# Autodesk Inventor assembly: Final assemply edit 2
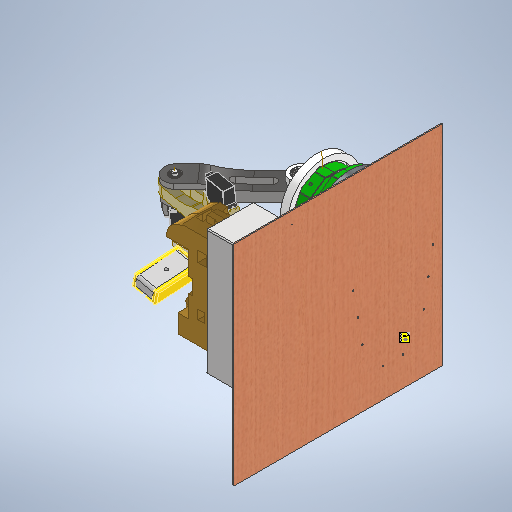
[picture p0: Inventor's stored thumbnail of the model, 512x512]
Saved by Autodesk Inventor 2025.2 (Build 292293000, 293)
## iProperties
Created: 2025-04-03
Part Number: Final assemply edit 2
Document SubType Name: Assembly
Designer: abdal
Author: abdal
## Documents named in this file (47)
- C:\Users\abdal\Desktop\FINAL MECHANICAL MOVMENT WITH STAND\Final assemply edit 2.iam
- C:\Users\abdal\Desktop\FINAL MECHANICAL MOVMENT WITH STAND\Link two .ipt
- C:\Users\abdal\Desktop\FINAL MECHANICAL MOVMENT WITH STAND\JIS B 1521 - 6800 10x19x5x1.72.ipt
- C:\Users\abdal\Desktop\FINAL MECHANICAL MOVMENT WITH STAND\DIN 472 - 19 x 1.ipt
- C:\Users\abdal\Desktop\FINAL MECHANICAL MOVMENT WITH STAND\Shaft between link2 and 3.ipt
- C:\Users\abdal\Desktop\FINAL MECHANICAL MOVMENT WITH STAND\DIN 471 - 10x1.ipt
- C:\Users\abdal\Desktop\FINAL MECHANICAL MOVMENT WITH STAND\Servo MG996R.ipt
- C:\Users\abdal\Desktop\FINAL MECHANICAL MOVMENT WITH STAND\Tower Pro MG90S Micro servo.ipt
- C:\Users\abdal\Desktop\FINAL MECHANICAL MOVMENT WITH STAND\Link Three .ipt
- C:\Users\abdal\Desktop\FINAL MECHANICAL MOVMENT WITH STAND\Link one1 .ipt
- C:\Users\abdal\Desktop\FINAL MECHANICAL MOVMENT WITH STAND\New End effector.ipt
- C:\Users\abdal\Desktop\FINAL MECHANICAL MOVMENT WITH STAND\Bidirectional shoulder.ipt
- C:\Users\abdal\Desktop\FINAL MECHANICAL MOVMENT WITH STAND\Rotating Plate edited.ipt
- C:\Users\abdal\Desktop\FINAL MECHANICAL MOVMENT WITH STAND\shatft extension.ipt
- C:\Users\abdal\Desktop\FINAL MECHANICAL MOVMENT WITH STAND\BS 292 Part 1 - 6001 - 12 x 28 x 8.ipt
- C:\Users\abdal\Desktop\FINAL MECHANICAL MOVMENT WITH STAND\DIN 471 - 12x1.ipt
- C:\Users\abdal\Desktop\FINAL MECHANICAL MOVMENT WITH STAND\DIN 472 - 28 x 1.5.ipt
- C:\Users\abdal\Desktop\FINAL MECHANICAL MOVMENT WITH STAND\Servo Horns.ipt
- C:\Users\abdal\Desktop\FINAL MECHANICAL MOVMENT WITH STAND\Printed Horn.ipt
- C:\Users\abdal\Desktop\FINAL MECHANICAL MOVMENT WITH STAND\JGY-370-1285_Motor_Assembly.ipt
- C:\Users\abdal\Desktop\FINAL MECHANICAL MOVMENT WITH STAND\Camera.ipt
- C:\Users\abdal\Desktop\FINAL MECHANICAL MOVMENT WITH STAND\BS 4174 - Type AB. No. 4 x 19 mm(1).ipt
- C:\Users\abdal\Desktop\FINAL MECHANICAL MOVMENT WITH STAND\BS 4174 - Type AB. No. 4 x 13 mm(1).ipt
- C:\Users\abdal\Desktop\FINAL MECHANICAL MOVMENT WITH STAND\BS 4174 - Type AB. No. 4 x 25 mm(1).ipt
- C:\Users\abdal\Desktop\FINAL MECHANICAL MOVMENT WITH STAND\scaled2.ipt
- C:\Users\abdal\Desktop\FINAL MECHANICAL MOVMENT WITH STAND\BASE.ipt
- C:\Users\abdal\Desktop\FINAL MECHANICAL MOVMENT WITH STAND\SHAFT.ipt
- C:\Users\abdal\Desktop\FINAL MECHANICAL MOVMENT WITH STAND\BS 5989_ Part 1 - 0 70 - 60x75x7.ipt
- C:\Users\abdal\Desktop\FINAL MECHANICAL MOVMENT WITH STAND\AS 1111 - M6 x 30.ipt
- C:\Users\abdal\Desktop\FINAL MECHANICAL MOVMENT WITH STAND\AS 1110 - M6 x 20.ipt
- C:\Users\abdal\Desktop\FINAL MECHANICAL MOVMENT WITH STAND\ANSI B18.2.4.2M - M6x1 - 10.ipt
- C:\Users\abdal\Desktop\FINAL MECHANICAL MOVMENT WITH STAND\AS 1427 - M2.5 x 12(5) I.ipt
- C:\Users\abdal\Desktop\FINAL MECHANICAL MOVMENT WITH STAND\holder for motor.ipt
- C:\Users\abdal\Desktop\FINAL MECHANICAL MOVMENT WITH STAND\DC Motor.ipt
- C:\Users\abdal\Desktop\FINAL MECHANICAL MOVMENT WITH STAND\Arduino_Mega.ipt
- C:\Users\abdal\Desktop\FINAL MECHANICAL MOVMENT WITH STAND\Breadboard Half.ipt
- C:\Users\abdal\Desktop\FINAL MECHANICAL MOVMENT WITH STAND\H-brug.ipt
- C:\Users\abdal\Documents\Inventor\Content Center Files\R2025\en-US\BS 4183(2)\BS 4183 - M3 x 7(1) I.ipt
- C:\Users\abdal\Documents\Inventor\Content Center Files\R2025\en-US\BS 4183(2)\BS 4183 - M2.5 x 5(1) I.ipt
- C:\Users\abdal\Desktop\FINAL MECHANICAL MOVMENT WITH STAND\Product stand .ipt
- C:\Users\abdal\Documents\Inventor\Content Center Files\R2025\en-US\BS 4183(2)\BS 4183 - M5 x 20(1) I.ipt
- C:\Users\abdal\Desktop\FINAL MECHANICAL MOVMENT WITH STAND\plate .ipt
- C:\Users\abdal\Desktop\FINAL MECHANICAL MOVMENT WITH STAND\L joint .ipt
- C:\Users\abdal\Desktop\FINAL MECHANICAL MOVMENT WITH STAND\L joint _MIR.ipt
- C:\Users\abdal\Documents\Inventor\Content Center Files\R2025\en-US\BS 4183(2)\BS 4183 - M3 x 10(1) I.ipt
- C:\Users\abdal\Documents\Inventor\Content Center Files\R2025\en-US\BS 4183(2)\BS 4183 - M3 x 8(1) I.ipt
- C:\Users\abdal\Desktop\FINAL MECHANICAL MOVMENT WITH STAND\casting pattern\casting pattern\casting pattern.iam
## Components (120 placed, 46 different names)
1. Link two :1 — Mate:1, Mate:2, Mate:5, Mate:6, Mate:15, Mate:19, Mate:35, Mate:36, Mate:37, Mate:74, Mate:85, Mate:86
2. JIS B 1521 6800 10x19x5:1 — Mate:1, Mate:2, Mate:3, Mate:4, Mate:7, Mate:10
3. JIS B 1521 6800 10x19x5:2 — Mate:5, Mate:8, Mate:12
4. DIN 472 19 x 1:1 — Mate:3, Mate:4
5. Shaft between link2 and 3:1 — Mate:6, Mate:7, Mate:8, Mate:9, Mate:11, Mate:13, Mate:18, Mate:38, Mate:84, Mate:93
6. DIN 471 10x1:1 — Mate:9, Mate:10
7. DIN 471 10x1:2 — Mate:11, Mate:12
8. Servo MG996R:1 — Mate:13, Mate:15, Mate:82, Mate:83, Mate:85, Mate:86, Flush:14, Flush:15, Flush:16, Flush:17, Mate:100, Mate:101, Mate:102, Mate:103
9. Tower Pro MG90S Micro servo:1 — Mate:16, Mate:17, Flush:1, Mate:40, Mate:41
10. Link Three :1 — Mate:16, Mate:17, Flush:1, Mate:18, Mate:19, Mate:38, Flush:28, Flush:29, Mate:156, Mate:157
11. Link one1 :1 — Mate:33, Mate:34, Mate:36, Mate:50, Mate:51, Mate:63, Mate:78, Mate:79, Mate:98, Mate:99
12. Servo MG996R:2 — Mate:67, Mate:68, Mate:78, Mate:79, Flush:10, Flush:11, Flush:12, Flush:13, Mate:96, Mate:97
13. Shaft between link2 and 3:2 — Mate:20, Mate:21, Mate:22, Mate:23, Mate:24, Mate:26, Mate:31, Mate:34, Mate:35, Mate:37, Mate:75, Mate:74, Mate:76, Mate:92
14. DIN 471 10x1:3 — Mate:24, Mate:25
15. DIN 471 10x1:4 — Mate:26, Mate:27
16. JIS B 1521 6800 10x19x5:3 — Mate:20, Mate:21, Mate:27, Mate:32, Mate:33
17. JIS B 1521 6800 10x19x5:4 — Mate:22, Mate:23, Mate:25
18. DIN 472 19 x 1:2 — Mate:31, Mate:32
19. New End effector:1 — Flush:6, Flush:8, Flush:9, Mate:94, Mate:95, Mate:176
20. Bidirectional shoulder:1 — Mate:40, Mate:41, Mate:94, Mate:95, Mate:176
21. Rotating Plate edited:1 — Mate:49, Mate:52, Mate:53, Mate:56, Mate:57, Mate:63, Mate:91, Flush:18, Flush:19, Flush:20, Flush:21, Mate:104, Mate:105, Mate:106, Mate:107, Mate:119, Flush:27, Mate:138, Mate:139, Mate:140, Mate:141, Mate:142, Mate:143
22. shatft extension:1 — Mate:49, Mate:50, Mate:51, Mate:54, Mate:58, Mate:60, Mate:62, Mate:89, Mate:90
23. BS 292: Part 1 (I) (Metric) 6001 - 12 x 28 x 8:1 — Mate:56, Mate:57, Mate:59, Mate:60, Mate:61
24. BS 292: Part 1 (I) (Metric) 6001 - 12 x 28 x 8:2 — Mate:52, Mate:53, Mate:55
25. DIN 471 12x1:1 — Mate:61, Mate:62
26. DIN 472 28 x 1.5:1 — Mate:58, Mate:59
27. DIN 472 28 x 1.5:2 — Mate:54, Mate:55
28. Servo Horns:1 — Mate:67, Mate:68, Mate:69, Mate:70
29. Printed Horn:1 — Mate:69, Mate:70, Mate:75, Mate:76, Mate:92
30. Servo Horns:2 — Mate:82, Mate:83
31. Printed Horn:2 — Mate:84, Mate:93
32. JGY-370-1285_Motor_Assembly:1 — Mate:89, Mate:90, Mate:91, Flush:22, Flush:23, Flush:24, Flush:25, Mate:108, Mate:109, Mate:110, Mate:111
33. Camera:1 — Flush:6, Flush:8, Flush:9, Flush:26, Mate:112
34. BS 4174 80° Cross Recessed Flat Countersunk Head Tapping Screw - Type AB - Metric Type AB. No. 4 x 19 mm:1 — Flush:10, Mate:98
35. BS 4174 80° Cross Recessed Flat Countersunk Head Tapping Screw - Type AB - Metric Type AB. No. 4 x 19 mm:2 — Flush:11, Mate:99
36. BS 4174 80° Cross Recessed Flat Countersunk Head Tapping Screw - Type AB - Metric Type AB. No. 4 x 19 mm:3 — Flush:12, Mate:96
37. BS 4174 80° Cross Recessed Flat Countersunk Head Tapping Screw - Type AB - Metric Type AB. No. 4 x 19 mm:4 — Flush:13, Mate:97
38. BS 4174 80° Cross Recessed Flat Countersunk Head Tapping Screw - Type AB - Metric Type AB. No. 4 x 19 mm:5 — Flush:14, Mate:103
39. BS 4174 80° Cross Recessed Flat Countersunk Head Tapping Screw - Type AB - Metric Type AB. No. 4 x 19 mm:6 — Flush:15, Mate:102
40. BS 4174 80° Cross Recessed Flat Countersunk Head Tapping Screw - Type AB - Metric Type AB. No. 4 x 19 mm:7 — Flush:17, Mate:100
41. BS 4174 80° Cross Recessed Flat Countersunk Head Tapping Screw - Type AB - Metric Type AB. No. 4 x 19 mm:8 — Flush:16, Mate:101
42. BS 4174 80° Cross Recessed Flat Countersunk Head Tapping Screw - Type AB - Metric Type AB. No. 4 x 13 mm:1 — Flush:18, Mate:106
43. BS 4174 80° Cross Recessed Flat Countersunk Head Tapping Screw - Type AB - Metric Type AB. No. 4 x 13 mm:2 — Flush:19, Mate:104
44. BS 4174 80° Cross Recessed Flat Countersunk Head Tapping Screw - Type AB - Metric Type AB. No. 4 x 13 mm:3 — Flush:21, Mate:105
45. BS 4174 80° Cross Recessed Flat Countersunk Head Tapping Screw - Type AB - Metric Type AB. No. 4 x 13 mm:4 — Flush:20, Mate:107
46. BS 4174 80° Cross Recessed Flat Countersunk Head Tapping Screw - Type AB - Metric Type AB. No. 4 x 13 mm:5 — Flush:22, Mate:109
47. BS 4174 80° Cross Recessed Flat Countersunk Head Tapping Screw - Type AB - Metric Type AB. No. 4 x 13 mm:6 — Flush:24, Mate:111
48. BS 4174 80° Cross Recessed Flat Countersunk Head Tapping Screw - Type AB - Metric Type AB. No. 4 x 13 mm:7 — Flush:25, Mate:110
49. BS 4174 80° Cross Recessed Flat Countersunk Head Tapping Screw - Type AB - Metric Type AB. No. 4 x 13 mm:8 — Flush:23, Mate:108
50. BS 4174 80° Cross Recessed Flat Countersunk Head Tapping Screw - Type AB - Metric Type AB. No. 4 x 25 mm:1 — Flush:26, Mate:112
51. scaled2:1 — Mate:116, Mate:117, Mate:120, Mate:125, Mate:126, Mate:127, Mate:128, Mate:129, Mate:130, Mate:131, Mate:132, Mate:133, Mate:134, Mate:135, Mate:136, Mate:137
52. BASE:1 — Mate:115, Mate:116, Mate:117, Mate:121, Mate:125, Mate:145, Mate:147, Mate:149, Mate:151, Mate:153, Mate:155, Mate:158, Mate:163, Mate:164, Mate:165, Mate:167, Mate:168, Mate:169, Flush:30, Flush:34, Mate:177, Mate:178, Mate:180, Mate:181, Mate:182, Flush:36, Flush:37, Mate:186, Mate:188, Mate:189, Mate:190, Mate:191, Mate:192, Mate:193, Mate:194, Mate:195, Mate:196, Mate:197, Mate:198, Mate:199, Mate:200, Mate:201, Mate:202, Mate:203, Mate:204, Mate:205, Mate:206, Flush:38, Mate:212, Mate:217, Mate:218, Mate:220, Mate:222
53. SHAFT:1 — Mate:115, Mate:119, Mate:122, Mate:123, Mate:124, Flush:27, Mate:162
54. BS 5989: Part 1 (Metric) 0 70 - 60x75x7:1 — Mate:120, Mate:121, Mate:122
55. BS 5989: Part 1 (Metric) 0 70 - 60x75x7:2 — Mate:123, Mate:124
56. AS 1111 - Metric M6 x 30:1 — Mate:126, Mate:127, Mate:154
57. AS 1111 - Metric M6 x 30:2 — Mate:132, Mate:133, Mate:148
58. AS 1111 - Metric M6 x 30:3 — Mate:128, Mate:137, Mate:144
59. AS 1111 - Metric M6 x 30:4 — Mate:129, Mate:136, Mate:150
60. AS 1111 - Metric M6 x 30:5 — Mate:131, Mate:135, Mate:152
61. AS 1111 - Metric M6 x 30:6 — Mate:130, Mate:134, Mate:146
62. AS 1110 - Metric M6 x 20:1 — Mate:138, Mate:143
63. AS 1110 - Metric M6 x 20:2 — Mate:140, Mate:141
64. AS 1110 - Metric M6 x 20:3 — Mate:139, Mate:142
65. ANSI B18.2.4.2M M6x1:1 — Mate:144, Mate:145
66. ANSI B18.2.4.2M M6x1:2 — Mate:146, Mate:147
67. ANSI B18.2.4.2M M6x1:3 — Mate:148, Mate:149
68. ANSI B18.2.4.2M M6x1:4 — Mate:150, Mate:151
69. ANSI B18.2.4.2M M6x1:5 — Mate:152, Mate:153
70. ANSI B18.2.4.2M M6x1:6 — Mate:154, Mate:155
71. AS 1427 H - Metric M2.5 x 12:1 — Flush:28, Mate:157
72. AS 1427 H - Metric M2.5 x 12:2 — Flush:29, Mate:156
73. holder for motor:1 — Mate:158, Mate:159, Mate:160, Mate:161, Mate:163, Mate:164, Mate:166, Mate:170, Mate:171, Mate:172
74. DC Motor:1 — Mate:159, Mate:160, Mate:161, Mate:162
75. BS 4174 80° Cross Recessed Flat Countersunk Head Tapping Screw - Type AB - Metric Type AB. No. 4 x 13 mm:9 — Mate:165, Mate:166
76. BS 4174 80° Cross Recessed Flat Countersunk Head Tapping Screw - Type AB - Metric Type AB. No. 4 x 13 mm:10 — Mate:168, Mate:171
77. BS 4174 80° Cross Recessed Flat Countersunk Head Tapping Screw - Type AB - Metric Type AB. No. 4 x 13 mm:11 — Mate:169, Mate:172
78. BS 4174 80° Cross Recessed Flat Countersunk Head Tapping Screw - Type AB - Metric Type AB. No. 4 x 13 mm:12 — Mate:167, Mate:170
79. Arduino_Mega:1 — Mate:177, Mate:178, Mate:188, Mate:207, Mate:208, Mate:209, Mate:210
80. Breadboard Half:1 — Mate:180, Mate:181
81. H-brug:1 — Mate:182, Flush:36, Mate:185, Mate:189, Mate:190
82. H-brug:2 — Flush:37, Mate:185, Mate:186
83. BS 4183 Cross Recessed Flat Countersunk Head Machine Screw - Metric M3 x 7:1 — Mate:191, Mate:192
84. BS 4183 Cross Recessed Flat Countersunk Head Machine Screw - Metric M3 x 7:2 — Mate:193, Mate:194
85. BS 4183 Cross Recessed Flat Countersunk Head Machine Screw - Metric M3 x 7:3 — Mate:195, Mate:201
86. BS 4183 Cross Recessed Flat Countersunk Head Machine Screw - Metric M3 x 7:4 — Mate:196, Mate:204
87. BS 4183 Cross Recessed Flat Countersunk Head Machine Screw - Metric M3 x 7:5 — Mate:197, Mate:202
88. BS 4183 Cross Recessed Flat Countersunk Head Machine Screw - Metric M3 x 7:6 — Mate:199, Mate:203
89. BS 4183 Cross Recessed Flat Countersunk Head Machine Screw - Metric M3 x 7:7 — Mate:200, Mate:206
90. BS 4183 Cross Recessed Flat Countersunk Head Machine Screw - Metric M3 x 7:8 — Mate:198, Mate:205
91. BS 4183 Cross Recessed Flat Countersunk Head Machine Screw - Metric M2.5 x 5:1 — Mate:207, Mate:210
92. BS 4183 Cross Recessed Flat Countersunk Head Machine Screw - Metric M2.5 x 5:2 — Mate:208, Mate:209
93. Product stand :1 — Flush:38, Mate:212, Mate:213, Mate:214, Mate:215, Flush:40, Flush:41, Mate:255, Mate:257
94. BS 4183 Cross Recessed Flat Countersunk Head Machine Screw - Metric M5 x 20:1 — Mate:213, Mate:214
95. plate :1 — Mate:215, Flush:40, Flush:41, Mate:216, Mate:219, Mate:221
96. L joint :1 — Mate:219, Mate:220, Mate:225, Mate:226, Mate:247, Mate:248
97. L joint :2 — Mate:216, Mate:217, Mate:218, Mate:223, Mate:224, Mate:249, Mate:250
98. L joint _MIR:1 — Mate:230, Mate:235, Mate:251, Mate:252
99. L joint _MIR:2 — Mate:231, Mate:234, Mate:253, Mate:254
100. L joint _MIR:3 — Mate:232, Mate:233, Mate:239, Mate:240
101. BS 4183 Cross Recessed Flat Countersunk Head Machine Screw - Metric M3 x 8:2 — Mate:223, Mate:224
102. BS 4183 Cross Recessed Flat Countersunk Head Machine Screw - Metric M3 x 8:1 — Mate:225, Mate:226
103. BS 4183 Cross Recessed Flat Countersunk Head Machine Screw - Metric M3 x 8:3 — Mate:229, Mate:238
104. BS 4183 Cross Recessed Flat Countersunk Head Machine Screw - Metric M3 x 8:4 — Mate:228, Mate:237
105. BS 4183 Cross Recessed Flat Countersunk Head Machine Screw - Metric M3 x 8:5 — Mate:227, Mate:236
106. BS 4183 Cross Recessed Flat Countersunk Head Machine Screw - Metric M3 x 8:6 — Mate:230, Mate:235
107. BS 4183 Cross Recessed Flat Countersunk Head Machine Screw - Metric M3 x 8:7 — Mate:231, Mate:234
108. BS 4183 Cross Recessed Flat Countersunk Head Machine Screw - Metric M3 x 8:8 — Mate:232, Mate:233
109. BS 4183 Cross Recessed Flat Countersunk Head Machine Screw - Metric M3 x 10:1 — Mate:239, Mate:240
110. BS 4183 Cross Recessed Flat Countersunk Head Machine Screw - Metric M3 x 10:2 — Mate:253, Mate:254
111. BS 4183 Cross Recessed Flat Countersunk Head Machine Screw - Metric M3 x 10:3 — Mate:251, Mate:252
112. BS 4183 Cross Recessed Flat Countersunk Head Machine Screw - Metric M3 x 10:4 — Mate:247, Mate:248
113. BS 4183 Cross Recessed Flat Countersunk Head Machine Screw - Metric M3 x 10:5 — Mate:249, Mate:250
114. BS 4183 Cross Recessed Flat Countersunk Head Machine Screw - Metric M3 x 10:6 — Mate:241, Mate:242
115. BS 4183 Cross Recessed Flat Countersunk Head Machine Screw - Metric M3 x 10:7 — Mate:243, Mate:244
116. BS 4183 Cross Recessed Flat Countersunk Head Machine Screw - Metric M3 x 10:8 — Mate:245, Mate:246
117. casting pattern:1 [sub-assembly] — Mate:255, Mate:256, Mate:257
118. L joint :3 — Mate:221, Mate:222, Mate:227, Mate:236, Mate:241, Mate:242
119. L joint :4 — Mate:228, Mate:237, Mate:243, Mate:244
120. L joint :5 — Mate:229, Mate:238, Mate:245, Mate:246
## Component patterns: (3 elements, first: L joint :3)
## Relationships (256: Mate 225, Flush 31)
- Mate:1: Link two :1 ↔ JIS B 1521 6800 10x19x5:1
- Mate:2: Link two :1 ↔ JIS B 1521 6800 10x19x5:1
- Mate:3: JIS B 1521 6800 10x19x5:1 ↔ DIN 472 19 x 1:1
- Mate:4: JIS B 1521 6800 10x19x5:1 ↔ DIN 472 19 x 1:1
- Mate:5: Link two :1 ↔ JIS B 1521 6800 10x19x5:2
- Mate:6: Link two :1 ↔ Shaft between link2 and 3:1
- Mate:7: JIS B 1521 6800 10x19x5:1 ↔ Shaft between link2 and 3:1
- Mate:8: JIS B 1521 6800 10x19x5:2 ↔ Shaft between link2 and 3:1
- Mate:9: Shaft between link2 and 3:1 ↔ DIN 471 10x1:1
- Mate:10: JIS B 1521 6800 10x19x5:1 ↔ DIN 471 10x1:1
- Mate:11: Shaft between link2 and 3:1 ↔ DIN 471 10x1:2
- Mate:12: JIS B 1521 6800 10x19x5:2 ↔ DIN 471 10x1:2
- Mate:13: Shaft between link2 and 3:1 ↔ Servo MG996R:1
- Mate:15: Link two :1 ↔ Servo MG996R:1
- Mate:16: Tower Pro MG90S Micro servo:1 ↔ Link Three :1
- Mate:17 (3.925 mm): Tower Pro MG90S Micro servo:1 ↔ Link Three :1
- Flush:1 (-7.189 mm): Tower Pro MG90S Micro servo:1 ↔ Link Three :1
- Mate:18: Shaft between link2 and 3:1 ↔ Link Three :1
- Mate:19 (1.5 mm): Link two :1 ↔ Link Three :1
- Mate:20: Shaft between link2 and 3:2 ↔ JIS B 1521 6800 10x19x5:3
- Mate:21: Shaft between link2 and 3:2 ↔ JIS B 1521 6800 10x19x5:3
- Mate:22: Shaft between link2 and 3:2 ↔ JIS B 1521 6800 10x19x5:4
- Mate:23: Shaft between link2 and 3:2 ↔ JIS B 1521 6800 10x19x5:4
- Mate:24: Shaft between link2 and 3:2 ↔ DIN 471 10x1:3
- Mate:25: DIN 471 10x1:3 ↔ JIS B 1521 6800 10x19x5:4
- Mate:26: Shaft between link2 and 3:2 ↔ DIN 471 10x1:4
- Mate:27: DIN 471 10x1:4 ↔ JIS B 1521 6800 10x19x5:3
- Mate:31: Shaft between link2 and 3:2 ↔ DIN 472 19 x 1:2
- Mate:32: JIS B 1521 6800 10x19x5:3 ↔ DIN 472 19 x 1:2
- Mate:33: Link one1 :1 ↔ JIS B 1521 6800 10x19x5:3
- Mate:34: Link one1 :1 ↔ Shaft between link2 and 3:2
- Mate:35: Link two :1 ↔ Shaft between link2 and 3:2
- Mate:36 (1 mm): Link two :1 ↔ Link one1 :1
- Mate:37: Link two :1 ↔ Shaft between link2 and 3:2
- Mate:38: Shaft between link2 and 3:1 ↔ Link Three :1
- Mate:40: Tower Pro MG90S Micro servo:1 ↔ Bidirectional shoulder:1
- Mate:41: Tower Pro MG90S Micro servo:1 ↔ Bidirectional shoulder:1
- Mate:49: Rotating Plate edited:1 ↔ shatft extension:1
- Mate:50: Link one1 :1 ↔ shatft extension:1
- Mate:51: Link one1 :1 ↔ shatft extension:1
- Mate:52: Rotating Plate edited:1 ↔ BS 292: Part 1 (I) (Metric) 6001 - 12 x 28 x 8:2
- Mate:53: Rotating Plate edited:1 ↔ BS 292: Part 1 (I) (Metric) 6001 - 12 x 28 x 8:2
- Mate:54: shatft extension:1 ↔ DIN 472 28 x 1.5:2
- Mate:55: BS 292: Part 1 (I) (Metric) 6001 - 12 x 28 x 8:2 ↔ DIN 472 28 x 1.5:2
- Mate:56: Rotating Plate edited:1 ↔ BS 292: Part 1 (I) (Metric) 6001 - 12 x 28 x 8:1
- Mate:57: Rotating Plate edited:1 ↔ BS 292: Part 1 (I) (Metric) 6001 - 12 x 28 x 8:1
- Mate:58: shatft extension:1 ↔ DIN 472 28 x 1.5:1
- Mate:59: BS 292: Part 1 (I) (Metric) 6001 - 12 x 28 x 8:1 ↔ DIN 472 28 x 1.5:1
- Mate:60: shatft extension:1 ↔ BS 292: Part 1 (I) (Metric) 6001 - 12 x 28 x 8:1
- Mate:61: BS 292: Part 1 (I) (Metric) 6001 - 12 x 28 x 8:1 ↔ DIN 471 12x1:1
- Mate:62: shatft extension:1 ↔ DIN 471 12x1:1
- Mate:63 (0.5 mm): Link one1 :1 ↔ Rotating Plate edited:1
- Mate:67: Servo MG996R:2 ↔ Servo Horns:1
- Mate:68: Servo MG996R:2 ↔ Servo Horns:1
- Mate:69: Servo Horns:1 ↔ Printed Horn:1
- Mate:70: Servo Horns:1 ↔ Printed Horn:1
- Mate:75: Shaft between link2 and 3:2 ↔ Printed Horn:1
- Mate:74: Link two :1 ↔ Shaft between link2 and 3:2
- Mate:76: Shaft between link2 and 3:2 ↔ Printed Horn:1
- Mate:78: Link one1 :1 ↔ Servo MG996R:2
- Mate:79: Link one1 :1 ↔ Servo MG996R:2
- [Mate]: Servo Horns:2 ↔ Printed Horn:2
- [Mate]: Servo Horns:2 ↔ Printed Horn:2
- Mate:82: Servo MG996R:1 ↔ Servo Horns:2
- Mate:83: Servo MG996R:1 ↔ Servo Horns:2
- Mate:84: Shaft between link2 and 3:1 ↔ Printed Horn:2
- Mate:85: Link two :1 ↔ Servo MG996R:1
- Mate:86: Link two :1 ↔ Servo MG996R:1
- Mate:89: shatft extension:1 ↔ JGY-370-1285_Motor_Assembly:1
- Mate:90 (1.5 mm): shatft extension:1 ↔ JGY-370-1285_Motor_Assembly:1
- Mate:91: Rotating Plate edited:1 ↔ JGY-370-1285_Motor_Assembly:1
- Mate:92 (2.5 mm): Shaft between link2 and 3:2 ↔ Printed Horn:1
- Mate:93 (2.5 mm): Shaft between link2 and 3:1 ↔ Printed Horn:2
- Flush:6 (7.039 mm): New End effector:1 ↔ Camera:1
- Flush:8: New End effector:1 ↔ Camera:1
- Flush:9: New End effector:1 ↔ Camera:1
- Mate:94: New End effector:1 ↔ Bidirectional shoulder:1
- Mate:95: New End effector:1 ↔ Bidirectional shoulder:1
- Flush:10 (-0.586 mm): Servo MG996R:2 ↔ BS 4174 80° Cross Recessed Flat Countersunk Head Tapping Screw - Type AB - Metric Type AB. No. 4 x 19 mm:1
- Flush:11 (-0.586 mm): Servo MG996R:2 ↔ BS 4174 80° Cross Recessed Flat Countersunk Head Tapping Screw - Type AB - Metric Type AB. No. 4 x 19 mm:2
- Flush:12 (-0.586 mm): Servo MG996R:2 ↔ BS 4174 80° Cross Recessed Flat Countersunk Head Tapping Screw - Type AB - Metric Type AB. No. 4 x 19 mm:3
- Flush:13 (-0.586 mm): Servo MG996R:2 ↔ BS 4174 80° Cross Recessed Flat Countersunk Head Tapping Screw - Type AB - Metric Type AB. No. 4 x 19 mm:4
- Mate:96: Servo MG996R:2 ↔ BS 4174 80° Cross Recessed Flat Countersunk Head Tapping Screw - Type AB - Metric Type AB. No. 4 x 19 mm:3
- Mate:97: Servo MG996R:2 ↔ BS 4174 80° Cross Recessed Flat Countersunk Head Tapping Screw - Type AB - Metric Type AB. No. 4 x 19 mm:4
- Mate:98: Link one1 :1 ↔ BS 4174 80° Cross Recessed Flat Countersunk Head Tapping Screw - Type AB - Metric Type AB. No. 4 x 19 mm:1
- Mate:99: Link one1 :1 ↔ BS 4174 80° Cross Recessed Flat Countersunk Head Tapping Screw - Type AB - Metric Type AB. No. 4 x 19 mm:2
- Flush:14 (-0.586 mm): Servo MG996R:1 ↔ BS 4174 80° Cross Recessed Flat Countersunk Head Tapping Screw - Type AB - Metric Type AB. No. 4 x 19 mm:5
- Flush:15 (-0.586 mm): Servo MG996R:1 ↔ BS 4174 80° Cross Recessed Flat Countersunk Head Tapping Screw - Type AB - Metric Type AB. No. 4 x 19 mm:6
- Flush:16 (-0.586 mm): Servo MG996R:1 ↔ BS 4174 80° Cross Recessed Flat Countersunk Head Tapping Screw - Type AB - Metric Type AB. No. 4 x 19 mm:8
- Flush:17 (-0.586 mm): Servo MG996R:1 ↔ BS 4174 80° Cross Recessed Flat Countersunk Head Tapping Screw - Type AB - Metric Type AB. No. 4 x 19 mm:7
- Mate:100: Servo MG996R:1 ↔ BS 4174 80° Cross Recessed Flat Countersunk Head Tapping Screw - Type AB - Metric Type AB. No. 4 x 19 mm:7
- Mate:101: Servo MG996R:1 ↔ BS 4174 80° Cross Recessed Flat Countersunk Head Tapping Screw - Type AB - Metric Type AB. No. 4 x 19 mm:8
- Mate:102: Servo MG996R:1 ↔ BS 4174 80° Cross Recessed Flat Countersunk Head Tapping Screw - Type AB - Metric Type AB. No. 4 x 19 mm:6
- Mate:103: Servo MG996R:1 ↔ BS 4174 80° Cross Recessed Flat Countersunk Head Tapping Screw - Type AB - Metric Type AB. No. 4 x 19 mm:5
- Flush:18 (-3.586 mm): Rotating Plate edited:1 ↔ BS 4174 80° Cross Recessed Flat Countersunk Head Tapping Screw - Type AB - Metric Type AB. No. 4 x 13 mm:1
- Flush:19 (-3.586 mm): Rotating Plate edited:1 ↔ BS 4174 80° Cross Recessed Flat Countersunk Head Tapping Screw - Type AB - Metric Type AB. No. 4 x 13 mm:2
- Flush:20 (-3.586 mm): Rotating Plate edited:1 ↔ BS 4174 80° Cross Recessed Flat Countersunk Head Tapping Screw - Type AB - Metric Type AB. No. 4 x 13 mm:4
- Flush:21 (-3.586 mm): Rotating Plate edited:1 ↔ BS 4174 80° Cross Recessed Flat Countersunk Head Tapping Screw - Type AB - Metric Type AB. No. 4 x 13 mm:3
- Mate:104: Rotating Plate edited:1 ↔ BS 4174 80° Cross Recessed Flat Countersunk Head Tapping Screw - Type AB - Metric Type AB. No. 4 x 13 mm:2
- Mate:105: Rotating Plate edited:1 ↔ BS 4174 80° Cross Recessed Flat Countersunk Head Tapping Screw - Type AB - Metric Type AB. No. 4 x 13 mm:3
- Mate:106: Rotating Plate edited:1 ↔ BS 4174 80° Cross Recessed Flat Countersunk Head Tapping Screw - Type AB - Metric Type AB. No. 4 x 13 mm:1
- Mate:107: Rotating Plate edited:1 ↔ BS 4174 80° Cross Recessed Flat Countersunk Head Tapping Screw - Type AB - Metric Type AB. No. 4 x 13 mm:4
- Flush:22 (-0.586 mm): JGY-370-1285_Motor_Assembly:1 ↔ BS 4174 80° Cross Recessed Flat Countersunk Head Tapping Screw - Type AB - Metric Type AB. No. 4 x 13 mm:5
- Flush:23 (-0.586 mm): JGY-370-1285_Motor_Assembly:1 ↔ BS 4174 80° Cross Recessed Flat Countersunk Head Tapping Screw - Type AB - Metric Type AB. No. 4 x 13 mm:8
- Flush:24 (-0.586 mm): JGY-370-1285_Motor_Assembly:1 ↔ BS 4174 80° Cross Recessed Flat Countersunk Head Tapping Screw - Type AB - Metric Type AB. No. 4 x 13 mm:6
- Flush:25 (-0.586 mm): JGY-370-1285_Motor_Assembly:1 ↔ BS 4174 80° Cross Recessed Flat Countersunk Head Tapping Screw - Type AB - Metric Type AB. No. 4 x 13 mm:7
- Mate:108: JGY-370-1285_Motor_Assembly:1 ↔ BS 4174 80° Cross Recessed Flat Countersunk Head Tapping Screw - Type AB - Metric Type AB. No. 4 x 13 mm:8
- Mate:109: JGY-370-1285_Motor_Assembly:1 ↔ BS 4174 80° Cross Recessed Flat Countersunk Head Tapping Screw - Type AB - Metric Type AB. No. 4 x 13 mm:5
- Mate:110: JGY-370-1285_Motor_Assembly:1 ↔ BS 4174 80° Cross Recessed Flat Countersunk Head Tapping Screw - Type AB - Metric Type AB. No. 4 x 13 mm:7
- Mate:111: JGY-370-1285_Motor_Assembly:1 ↔ BS 4174 80° Cross Recessed Flat Countersunk Head Tapping Screw - Type AB - Metric Type AB. No. 4 x 13 mm:6
- Flush:26 (-0.586 mm): Camera:1 ↔ BS 4174 80° Cross Recessed Flat Countersunk Head Tapping Screw - Type AB - Metric Type AB. No. 4 x 25 mm:1
- Mate:112: Camera:1 ↔ BS 4174 80° Cross Recessed Flat Countersunk Head Tapping Screw - Type AB - Metric Type AB. No. 4 x 25 mm:1
- Mate:115: BASE:1 ↔ SHAFT:1
- Mate:116: scaled2:1 ↔ BASE:1
- Mate:117: scaled2:1 ↔ BASE:1
- Mate:119: Rotating Plate edited:1 ↔ SHAFT:1
- Mate:120: scaled2:1 ↔ BS 5989: Part 1 (Metric) 0 70 - 60x75x7:1
- Mate:121: BASE:1 ↔ BS 5989: Part 1 (Metric) 0 70 - 60x75x7:1
- Mate:122: SHAFT:1 ↔ BS 5989: Part 1 (Metric) 0 70 - 60x75x7:1
- Mate:123: SHAFT:1 ↔ BS 5989: Part 1 (Metric) 0 70 - 60x75x7:2
- Mate:124: SHAFT:1 ↔ BS 5989: Part 1 (Metric) 0 70 - 60x75x7:2
- Mate:125: scaled2:1 ↔ BASE:1
- Flush:27 (7.5 mm): Rotating Plate edited:1 ↔ SHAFT:1
- Mate:126: scaled2:1 ↔ AS 1111 - Metric M6 x 30:1
- Mate:127: scaled2:1 ↔ AS 1111 - Metric M6 x 30:1
- Mate:128: scaled2:1 ↔ AS 1111 - Metric M6 x 30:3
- Mate:129: scaled2:1 ↔ AS 1111 - Metric M6 x 30:4
- Mate:130: scaled2:1 ↔ AS 1111 - Metric M6 x 30:6
- Mate:131: scaled2:1 ↔ AS 1111 - Metric M6 x 30:5
- Mate:132: scaled2:1 ↔ AS 1111 - Metric M6 x 30:2
- Mate:133: scaled2:1 ↔ AS 1111 - Metric M6 x 30:2
- Mate:134: scaled2:1 ↔ AS 1111 - Metric M6 x 30:6
- Mate:135: scaled2:1 ↔ AS 1111 - Metric M6 x 30:5
- Mate:136: scaled2:1 ↔ AS 1111 - Metric M6 x 30:4
- Mate:137: scaled2:1 ↔ AS 1111 - Metric M6 x 30:3
- Mate:138: Rotating Plate edited:1 ↔ AS 1110 - Metric M6 x 20:1
- Mate:139: Rotating Plate edited:1 ↔ AS 1110 - Metric M6 x 20:3
- Mate:140: Rotating Plate edited:1 ↔ AS 1110 - Metric M6 x 20:2
- Mate:141: Rotating Plate edited:1 ↔ AS 1110 - Metric M6 x 20:2
- Mate:142: Rotating Plate edited:1 ↔ AS 1110 - Metric M6 x 20:3
- Mate:143: Rotating Plate edited:1 ↔ AS 1110 - Metric M6 x 20:1
- Mate:144: AS 1111 - Metric M6 x 30:3 ↔ ANSI B18.2.4.2M M6x1:1
- Mate:145: BASE:1 ↔ ANSI B18.2.4.2M M6x1:1
- Mate:146: AS 1111 - Metric M6 x 30:6 ↔ ANSI B18.2.4.2M M6x1:2
- Mate:147: BASE:1 ↔ ANSI B18.2.4.2M M6x1:2
- Mate:148: AS 1111 - Metric M6 x 30:2 ↔ ANSI B18.2.4.2M M6x1:3
- Mate:149: BASE:1 ↔ ANSI B18.2.4.2M M6x1:3
- Mate:150: AS 1111 - Metric M6 x 30:4 ↔ ANSI B18.2.4.2M M6x1:4
- Mate:151: BASE:1 ↔ ANSI B18.2.4.2M M6x1:4
- Mate:152: AS 1111 - Metric M6 x 30:5 ↔ ANSI B18.2.4.2M M6x1:5
- Mate:153: BASE:1 ↔ ANSI B18.2.4.2M M6x1:5
- Mate:154: AS 1111 - Metric M6 x 30:1 ↔ ANSI B18.2.4.2M M6x1:6
- Mate:155: BASE:1 ↔ ANSI B18.2.4.2M M6x1:6
- Flush:28 (-1.5 mm): Link Three :1 ↔ AS 1427 H - Metric M2.5 x 12:1
- Flush:29 (-1.5 mm): Link Three :1 ↔ AS 1427 H - Metric M2.5 x 12:2
- Mate:156: Link Three :1 ↔ AS 1427 H - Metric M2.5 x 12:2
- Mate:157: Link Three :1 ↔ AS 1427 H - Metric M2.5 x 12:1
- Mate:158: BASE:1 ↔ holder for motor:1
- Mate:159: holder for motor:1 ↔ DC Motor:1
- Mate:160: holder for motor:1 ↔ DC Motor:1
- Mate:161: holder for motor:1 ↔ DC Motor:1
- Mate:162 (4.5 mm): SHAFT:1 ↔ DC Motor:1
- Mate:163: BASE:1 ↔ holder for motor:1
- Mate:164: BASE:1 ↔ holder for motor:1
- Mate:165: BASE:1 ↔ BS 4174 80° Cross Recessed Flat Countersunk Head Tapping Screw - Type AB - Metric Type AB. No. 4 x 13 mm:9
- Mate:166: holder for motor:1 ↔ BS 4174 80° Cross Recessed Flat Countersunk Head Tapping Screw - Type AB - Metric Type AB. No. 4 x 13 mm:9
- Mate:167: BASE:1 ↔ BS 4174 80° Cross Recessed Flat Countersunk Head Tapping Screw - Type AB - Metric Type AB. No. 4 x 13 mm:12
- Mate:168: BASE:1 ↔ BS 4174 80° Cross Recessed Flat Countersunk Head Tapping Screw - Type AB - Metric Type AB. No. 4 x 13 mm:10
- Mate:169: BASE:1 ↔ BS 4174 80° Cross Recessed Flat Countersunk Head Tapping Screw - Type AB - Metric Type AB. No. 4 x 13 mm:11
- Mate:170: holder for motor:1 ↔ BS 4174 80° Cross Recessed Flat Countersunk Head Tapping Screw - Type AB - Metric Type AB. No. 4 x 13 mm:12
- Mate:171: holder for motor:1 ↔ BS 4174 80° Cross Recessed Flat Countersunk Head Tapping Screw - Type AB - Metric Type AB. No. 4 x 13 mm:10
- Mate:172: holder for motor:1 ↔ BS 4174 80° Cross Recessed Flat Countersunk Head Tapping Screw - Type AB - Metric Type AB. No. 4 x 13 mm:11
- Flush:30: BASE:1
- Flush:34 (15 mm): BASE:1
- Mate:176: New End effector:1 ↔ Bidirectional shoulder:1
- Mate:177: BASE:1 ↔ Arduino_Mega:1
- Mate:178: BASE:1 ↔ Arduino_Mega:1
- Mate:180: BASE:1 ↔ Breadboard Half:1
- Mate:181: BASE:1 ↔ Breadboard Half:1
- Mate:182: BASE:1 ↔ H-brug:1
- Flush:36 (1 mm): BASE:1 ↔ H-brug:1
- Flush:37 (1 mm): BASE:1 ↔ H-brug:2
- Mate:185 (5 mm): H-brug:1 ↔ H-brug:2
- Mate:186: BASE:1 ↔ H-brug:2
- Mate:188: BASE:1 ↔ Arduino_Mega:1
- Mate:189: BASE:1 ↔ H-brug:1
- Mate:190: BASE:1 ↔ H-brug:1
- Mate:191: BASE:1 ↔ BS 4183 Cross Recessed Flat Countersunk Head Machine Screw - Metric M3 x 7:1
- Mate:192: BASE:1 ↔ BS 4183 Cross Recessed Flat Countersunk Head Machine Screw - Metric M3 x 7:1
- Mate:193: BASE:1 ↔ BS 4183 Cross Recessed Flat Countersunk Head Machine Screw - Metric M3 x 7:2
- Mate:194: BASE:1 ↔ BS 4183 Cross Recessed Flat Countersunk Head Machine Screw - Metric M3 x 7:2
- Mate:195: BASE:1 ↔ BS 4183 Cross Recessed Flat Countersunk Head Machine Screw - Metric M3 x 7:3
- Mate:196: BASE:1 ↔ BS 4183 Cross Recessed Flat Countersunk Head Machine Screw - Metric M3 x 7:4
- Mate:197: BASE:1 ↔ BS 4183 Cross Recessed Flat Countersunk Head Machine Screw - Metric M3 x 7:5
- Mate:198: BASE:1 ↔ BS 4183 Cross Recessed Flat Countersunk Head Machine Screw - Metric M3 x 7:8
- Mate:199: BASE:1 ↔ BS 4183 Cross Recessed Flat Countersunk Head Machine Screw - Metric M3 x 7:6
- Mate:200: BASE:1 ↔ BS 4183 Cross Recessed Flat Countersunk Head Machine Screw - Metric M3 x 7:7
- Mate:201: BASE:1 ↔ BS 4183 Cross Recessed Flat Countersunk Head Machine Screw - Metric M3 x 7:3
- Mate:202: BASE:1 ↔ BS 4183 Cross Recessed Flat Countersunk Head Machine Screw - Metric M3 x 7:5
- Mate:203: BASE:1 ↔ BS 4183 Cross Recessed Flat Countersunk Head Machine Screw - Metric M3 x 7:6
- Mate:204: BASE:1 ↔ BS 4183 Cross Recessed Flat Countersunk Head Machine Screw - Metric M3 x 7:4
- Mate:205: BASE:1 ↔ BS 4183 Cross Recessed Flat Countersunk Head Machine Screw - Metric M3 x 7:8
- Mate:206: BASE:1 ↔ BS 4183 Cross Recessed Flat Countersunk Head Machine Screw - Metric M3 x 7:7
- Mate:207: Arduino_Mega:1 ↔ BS 4183 Cross Recessed Flat Countersunk Head Machine Screw - Metric M2.5 x 5:1
- Mate:208: Arduino_Mega:1 ↔ BS 4183 Cross Recessed Flat Countersunk Head Machine Screw - Metric M2.5 x 5:2
- Mate:209: Arduino_Mega:1 ↔ BS 4183 Cross Recessed Flat Countersunk Head Machine Screw - Metric M2.5 x 5:2
- Mate:210: Arduino_Mega:1 ↔ BS 4183 Cross Recessed Flat Countersunk Head Machine Screw - Metric M2.5 x 5:1
- Flush:38: BASE:1 ↔ Product stand :1
- Mate:212: BASE:1 ↔ Product stand :1
- Mate:213: Product stand :1 ↔ BS 4183 Cross Recessed Flat Countersunk Head Machine Screw - Metric M5 x 20:1
- Mate:214: Product stand :1 ↔ BS 4183 Cross Recessed Flat Countersunk Head Machine Screw - Metric M5 x 20:1
- Mate:215: Product stand :1 ↔ plate :1
- Flush:40 (25 mm): Product stand :1 ↔ plate :1
- Flush:41 (25 mm): Product stand :1 ↔ plate :1
- Mate:216: plate :1 ↔ L joint :2
- Mate:217: BASE:1 ↔ L joint :2
- Mate:218 (15 mm): BASE:1 ↔ L joint :2
- Mate:219: plate :1 ↔ L joint :1
- Mate:220: BASE:1 ↔ L joint :1
- Mate:221: plate :1 ↔ L joint :3
- Mate:222: BASE:1 ↔ L joint :3
- Mate:223: L joint :2 ↔ BS 4183 Cross Recessed Flat Countersunk Head Machine Screw - Metric M3 x 8:2
- Mate:224: L joint :2 ↔ BS 4183 Cross Recessed Flat Countersunk Head Machine Screw - Metric M3 x 8:2
- Mate:225: L joint :1 ↔ BS 4183 Cross Recessed Flat Countersunk Head Machine Screw - Metric M3 x 8:1
- Mate:226: L joint :1 ↔ BS 4183 Cross Recessed Flat Countersunk Head Machine Screw - Metric M3 x 8:1
- Mate:227: BS 4183 Cross Recessed Flat Countersunk Head Machine Screw - Metric M3 x 8:5 ↔ L joint :3
- Mate:228: BS 4183 Cross Recessed Flat Countersunk Head Machine Screw - Metric M3 x 8:4 ↔ L joint :4
- Mate:229: BS 4183 Cross Recessed Flat Countersunk Head Machine Screw - Metric M3 x 8:3 ↔ L joint :5
- Mate:230: L joint _MIR:1 ↔ BS 4183 Cross Recessed Flat Countersunk Head Machine Screw - Metric M3 x 8:6
- Mate:231: L joint _MIR:2 ↔ BS 4183 Cross Recessed Flat Countersunk Head Machine Screw - Metric M3 x 8:7
- Mate:232: L joint _MIR:3 ↔ BS 4183 Cross Recessed Flat Countersunk Head Machine Screw - Metric M3 x 8:8
- Mate:233: L joint _MIR:3 ↔ BS 4183 Cross Recessed Flat Countersunk Head Machine Screw - Metric M3 x 8:8
- Mate:234: L joint _MIR:2 ↔ BS 4183 Cross Recessed Flat Countersunk Head Machine Screw - Metric M3 x 8:7
- Mate:235: L joint _MIR:1 ↔ BS 4183 Cross Recessed Flat Countersunk Head Machine Screw - Metric M3 x 8:6
- Mate:236: BS 4183 Cross Recessed Flat Countersunk Head Machine Screw - Metric M3 x 8:5 ↔ L joint :3
- Mate:237: BS 4183 Cross Recessed Flat Countersunk Head Machine Screw - Metric M3 x 8:4 ↔ L joint :4
- Mate:238: BS 4183 Cross Recessed Flat Countersunk Head Machine Screw - Metric M3 x 8:3 ↔ L joint :5
- Mate:239: L joint _MIR:3 ↔ BS 4183 Cross Recessed Flat Countersunk Head Machine Screw - Metric M3 x 10:1
- Mate:240: L joint _MIR:3 ↔ BS 4183 Cross Recessed Flat Countersunk Head Machine Screw - Metric M3 x 10:1
- Mate:241: BS 4183 Cross Recessed Flat Countersunk Head Machine Screw - Metric M3 x 10:6 ↔ L joint :3
- Mate:242: BS 4183 Cross Recessed Flat Countersunk Head Machine Screw - Metric M3 x 10:6 ↔ L joint :3
- Mate:243: BS 4183 Cross Recessed Flat Countersunk Head Machine Screw - Metric M3 x 10:7 ↔ L joint :4
- Mate:244: BS 4183 Cross Recessed Flat Countersunk Head Machine Screw - Metric M3 x 10:7 ↔ L joint :4
- Mate:245: BS 4183 Cross Recessed Flat Countersunk Head Machine Screw - Metric M3 x 10:8 ↔ L joint :5
- Mate:246: BS 4183 Cross Recessed Flat Countersunk Head Machine Screw - Metric M3 x 10:8 ↔ L joint :5
- Mate:247: L joint :1 ↔ BS 4183 Cross Recessed Flat Countersunk Head Machine Screw - Metric M3 x 10:4
- Mate:248: L joint :1 ↔ BS 4183 Cross Recessed Flat Countersunk Head Machine Screw - Metric M3 x 10:4
- Mate:249: L joint :2 ↔ BS 4183 Cross Recessed Flat Countersunk Head Machine Screw - Metric M3 x 10:5
- Mate:250: L joint :2 ↔ BS 4183 Cross Recessed Flat Countersunk Head Machine Screw - Metric M3 x 10:5
- Mate:251: L joint _MIR:1 ↔ BS 4183 Cross Recessed Flat Countersunk Head Machine Screw - Metric M3 x 10:3
- Mate:252: L joint _MIR:1 ↔ BS 4183 Cross Recessed Flat Countersunk Head Machine Screw - Metric M3 x 10:3
- Mate:253: L joint _MIR:2 ↔ BS 4183 Cross Recessed Flat Countersunk Head Machine Screw - Metric M3 x 10:2
- Mate:254: L joint _MIR:2 ↔ BS 4183 Cross Recessed Flat Countersunk Head Machine Screw - Metric M3 x 10:2
- Mate:255: Product stand :1 ↔ casting pattern:1
- Mate:256 (200 mm): casting pattern:1
- Mate:257: Product stand :1 ↔ casting pattern:1
## Named parameters: d89_d78 = 0 mm, d90_d79 = 0 mm
